# Autodesk Inventor assembly: endeffector motor assembly
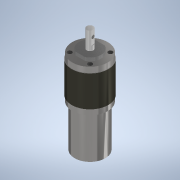
[picture p0: Inventor's stored thumbnail of the model, 180x180]
Saved by Autodesk Inventor 2020 (Build 240168000, 168)
## iProperties
Created: 2020-07-29
Part Number: endeffector motor assembly
Document SubType Name: Assembly
Designer: Vikki
Author: Vikki
## Documents named in this file (3)
- E:\project inventor pro\flipkart grid models\articulated arm\endeffector motor assembly.iam
- C:\Users\Vikki\AppData\Local\Temp\Temp1_end effector motor.zip\end effector motor\motor_body.ipt
- C:\Users\Vikki\AppData\Local\Temp\Temp1_end effector motor.zip\end effector motor\motor shaft.ipt
## Components (2 placed, 2 different names)
1. motor_body:1 — Mate:1, Mate:2
2. motor shaft:1 — Mate:1, Mate:2
## Relationships (2: Mate 2)
- Mate:1: motor_body:1 ↔ motor shaft:1
- Mate:2: motor_body:1 ↔ motor shaft:1
